# Autodesk Inventor assembly: LeftLowerArmUnit
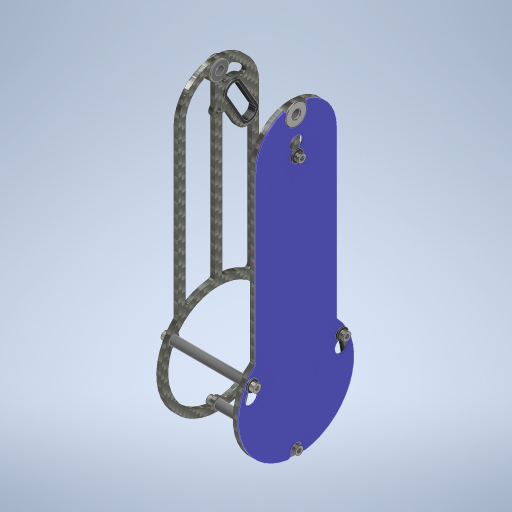
[picture p0: Inventor's stored thumbnail of the model, 512x512]
Saved by Autodesk Inventor 2024.2 (Build 282272000, 272)
## iProperties
Created: 2024-01-18
Part Number: LeftLowerArmUnit
Document SubType Name: Assembly
Designer: Masato Kubotera
Mass: 41.7513 g
Surface Area: 463.198 cm^2
Volume: 27.2767 cm^3
Author: Masato Kubotera
## Documents named in this file (13)
- C:\Users\masato\OneDrive - Chiba Institute of Technology\CIT Brains\RoboCup2024\Mechanic\SUSTAINA-OP2-DEV\NativeFiles\Boby\UpperLimb\LowerArms\LeftLowerArmUnit.iam
- C:\Users\masato\OneDrive - Chiba Institute of Technology\CIT Brains\RoboCup2024\Mechanic\SUSTAINA-OP2-DEV\NativeFiles\Boby\UpperLimb\LowerArms\LowerArmFrame.ipt
- C:\Users\masato\OneDrive - Chiba Institute of Technology\CIT Brains\RoboCup2024\Mechanic\SUSTAINA-OP2-DEV\NativeFiles\Boby\COTS\Bushes\GFM-0608-04.ipt
- C:\Users\masato\OneDrive - Chiba Institute of Technology\CIT Brains\RoboCup2024\Mechanic\SUSTAINA-OP2-DEV\NativeFiles\Boby\COTS\Washers\Metal\UUW-0614-05H.ipt
- C:\Users\masato\OneDrive - Chiba Institute of Technology\CIT Brains\RoboCup2024\Mechanic\SUSTAINA-OP2-DEV\NativeFiles\Boby\CommonDesignedComponents\SliderProtectionFrame.ipt
- C:\Users\masato\OneDrive - Chiba Institute of Technology\CIT Brains\RoboCup2024\Mechanic\SUSTAINA-OP2-DEV\NativeFiles\Boby\COTS\Spacers\AR-350B.ipt
- C:\Users\masato\OneDrive - Chiba Institute of Technology\CIT Brains\RoboCup2024\Mechanic\SUSTAINA-OP2-DEV\NativeFiles\Boby\COTS\Screws\CapScrew\UC-0308.ipt
- C:\Users\masato\OneDrive - Chiba Institute of Technology\CIT Brains\RoboCup2024\Mechanic\SUSTAINA-OP2-DEV\NativeFiles\Boby\COTS\Screws\CapScrew\UC-0310.ipt
- C:\Users\masato\OneDrive - Chiba Institute of Technology\CIT Brains\RoboCup2024\Mechanic\SUSTAINA-OP2-DEV\NativeFiles\Boby\COTS\Bushes\L3040-8110TB.ipt
- C:\Users\masato\OneDrive - Chiba Institute of Technology\CIT Brains\RoboCup2024\Mechanic\SUSTAINA-OP2-DEV\NativeFiles\Boby\UpperLimb\LowerArms\LowerArmColorMarker.ipt
- C:\Users\masato\OneDrive - Chiba Institute of Technology\CIT Brains\RoboCup2024\Mechanic\SUSTAINA-OP2-DEV\NativeFiles\Boby\COTS\Screws\CapScrew\UC-0306.ipt
- C:\Users\masato\OneDrive - Chiba Institute of Technology\CIT Brains\RoboCup2024\Mechanic\SUSTAINA-OP2-DEV\NativeFiles\Boby\COTS\Nuts\UNT-03-3.ipt
- C:\Users\masato\OneDrive - Chiba Institute of Technology\CIT Brains\RoboCup2024\Mechanic\SUSTAINA-OP2-DEV\NativeFiles\Boby\COTS\Washers\Resin\TT-0614-05.ipt
## Components (24 placed, 12 different names)
1. UNT-03-3:1 — Insert:29
2. LowerArmFrame:1 — Mate:1, Symmetry:1, Angle:1, Insert:1, Insert:3, Insert:7, Insert:8, Insert:11, Insert:12, Insert:13, Insert:17, Insert:18, Insert:19
3. LowerArmFrame:2 — Insert:2, Insert:4, Insert:14, Insert:15, Insert:16, Insert:20, Insert:21, Insert:22, Symmetry:1, Insert:28, Insert:29
4. SliderProtectionFrame:1 — Insert:7, Insert:8
5. LowerArmColorMarker:1 — Insert:25, Insert:26
6. GFM-0608-04:1 — Insert:1
7. GFM-0608-04:2 — Insert:2
8. L3040-8110TB:1 — Insert:21, Insert:23, Insert:25
9. L3040-8110TB:2 — Insert:22, Insert:24, Insert:26
10. L3040-8110TB:3 — Insert:28
11. TT-0614-05:2 — Insert:3, Insert:5
12. TT-0614-05:1 — Insert:4, Insert:6
13. UUW-0614-05H:1 — Insert:5
14. UUW-0614-05H:2 — Insert:6
15. AR-350B:1 — Insert:11, Insert:14
16. AR-350B:2 — Insert:12, Insert:15
17. AR-350B:3 — Insert:13, Insert:16
18. UC-0306:1
19. UC-0308:1 — Insert:17
20. UC-0308:2 — Insert:18
21. UC-0308:3 — Insert:19
22. UC-0308:4 — Insert:20
23. UC-0310:1 — Insert:23
24. UC-0310:2 — Insert:24
## Relationships (30: Insert 27, Mate 1, Symmetry 1, Angle 1)
- Mate:1: LowerArmFrame:1
- Symmetry:1: LowerArmFrame:1 ↔ LowerArmFrame:2
- Angle:1 (0 deg): LowerArmFrame:1
- Insert:1: LowerArmFrame:1 ↔ GFM-0608-04:1
- Insert:2: LowerArmFrame:2 ↔ GFM-0608-04:2
- Insert:3: LowerArmFrame:1 ↔ TT-0614-05:2
- Insert:4: LowerArmFrame:2 ↔ TT-0614-05:1
- Insert:5: TT-0614-05:2 ↔ UUW-0614-05H:1
- Insert:6: TT-0614-05:1 ↔ UUW-0614-05H:2
- Insert:7: LowerArmFrame:1 ↔ SliderProtectionFrame:1
- Insert:8: LowerArmFrame:1 ↔ SliderProtectionFrame:1
- Insert:11: LowerArmFrame:1 ↔ AR-350B:1
- Insert:12: LowerArmFrame:1 ↔ AR-350B:2
- Insert:13: LowerArmFrame:1 ↔ AR-350B:3
- Insert:14: LowerArmFrame:2 ↔ AR-350B:1
- Insert:15: LowerArmFrame:2 ↔ AR-350B:2
- Insert:16: LowerArmFrame:2 ↔ AR-350B:3
- Insert:17: LowerArmFrame:1 ↔ UC-0308:1
- Insert:18: LowerArmFrame:1 ↔ UC-0308:2
- Insert:19: LowerArmFrame:1 ↔ UC-0308:3
- Insert:20: LowerArmFrame:2 ↔ UC-0308:4
- Insert:21: LowerArmFrame:2 ↔ L3040-8110TB:1
- Insert:22: LowerArmFrame:2 ↔ L3040-8110TB:2
- Insert:23: L3040-8110TB:1 ↔ UC-0310:1
- Insert:24: L3040-8110TB:2 ↔ UC-0310:2
- Insert:25: LowerArmColorMarker:1 ↔ L3040-8110TB:1
- Insert:26: LowerArmColorMarker:1 ↔ L3040-8110TB:2
- [Insert]: L3040-8110TB:3 ↔ UC-0306:1
- Insert:28: LowerArmFrame:2 ↔ L3040-8110TB:3
- Insert:29: UNT-03-3:1 ↔ LowerArmFrame:2
## Named parameters: d31_d27 = 0 mm
